# Autodesk Inventor assembly: wheel assembly
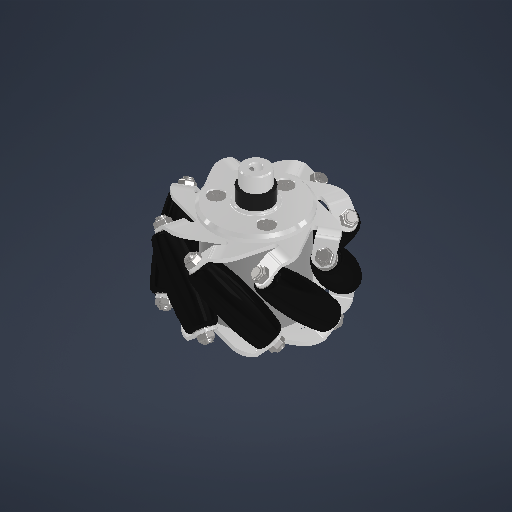
[picture p0: Inventor's stored thumbnail of the model, 512x512]
Saved by Autodesk Inventor 2025 (Build 290162000, 162)
## iProperties
Created: 2023-06-24
Part Number: wheel assembly
Document SubType Name: Assembly
Designer: khrip
Mass: 249.664 g
Surface Area: 386.365 cm^2
Volume: 54.6179 cm^3
Density: 4.5711 g/cm^3
Author: khrip
## Documents named in this file (9)
- H:\Botik\Chassis\UnsprungUnits\Wheels\wheel assembly.iam
- H:\Botik\Chassis\UnsprungUnits\Wheels\Parts\wheelHub.ipt
- H:\Botik\Chassis\UnsprungUnits\Wheels\wheelAss\Mecanum_Wheel_60mm_Right_ASM_AP214.iam
- H:\Botik\Chassis\UnsprungUnits\Wheels\Parts\washer.ipt
- C:\Users\khrip\Documents\Inventor\Content Center Files\R2025\ru-RU\GOST 17475-80 (2)\Винт 2.M4-6gx40 ГОСТ 17475-80.ipt
- C:\Users\khrip\Documents\Inventor\Content Center Files\R2025\ru-RU\GOST 17475-80 (2)\Винт 2.M3-6gx40 ГОСТ 17475-80.ipt
- C:\Users\khrip\Documents\Inventor\Content Center Files\R2025\ru-RU\GOST 11371-78  A\Шайба 3 ГОСТ 11371-78.ipt
- C:\Users\khrip\Documents\Inventor\Content Center Files\R2025\ru-RU\DIN 985\DIN 985 - M3.ipt
- H:\Botik\Chassis\UnsprungUnits\Wheels\Parts\fittingRingInstalled.ipt
## Components (14 placed, 8 different names)
1. wheelHub:1 — Совмещение:1, Совмещение:2, Совмещение:3, Совмещение:8, Совмещение:9, Совмещение:10, Совмещение:24, Совмещение:25
2. Mecanum_Wheel_60mm_Right_ASM_AP214:2 [sub-assembly] — Совмещение:1, Совмещение:2, Совмещение:3, Совмещение:4, Совмещение:5, Совмещение:6, Совмещение:12, Совмещение:14, Совмещение:16
3. washer:1 — Совмещение:4, Совмещение:5, Совмещение:6, Совмещение:7
4. Винт 2 ГОСТ 17475-80 M4 x 40:1 — Совмещение:7
5. Винт 2 ГОСТ 17475-80 M3 x 40:1 — Совмещение:8, Совмещение:13, Совмещение:19
6. Винт 2 ГОСТ 17475-80 M3 x 40:2 — Совмещение:9, Совмещение:11, Совмещение:21
7. Винт 2 ГОСТ 17475-80 M3 x 40:3 — Совмещение:10, Совмещение:15, Совмещение:17
8. Шайба  ГОСТ 11371-78 3,2:1 — Совмещение:11, Совмещение:12, Совмещение:22
9. Шайба  ГОСТ 11371-78 3,2:2 — Совмещение:13, Совмещение:14, Совмещение:20
10. Шайба  ГОСТ 11371-78 3,2:3 — Совмещение:15, Совмещение:16, Совмещение:18
11. DIN 985 - заменено на DIN EN ISO 10511 M3:1 — Совмещение:17, Совмещение:18
12. DIN 985 - заменено на DIN EN ISO 10511 M3:2 — Совмещение:19, Совмещение:20
13. DIN 985 - заменено на DIN EN ISO 10511 M3:3 — Совмещение:21, Совмещение:22
14. fittingRingInstalled:1 — Совмещение:24, Совмещение:25
## Relationships (24: Mate 24)
- Совмещение:1 [Mate]: wheelHub:1 ↔ Mecanum_Wheel_60mm_Right_ASM_AP214:2
- Совмещение:2 [Mate]: wheelHub:1 ↔ Mecanum_Wheel_60mm_Right_ASM_AP214:2
- Совмещение:3 [Mate]: wheelHub:1 ↔ Mecanum_Wheel_60mm_Right_ASM_AP214:2
- Совмещение:4 [Mate]: Mecanum_Wheel_60mm_Right_ASM_AP214:2 ↔ washer:1
- Совмещение:5 [Mate]: Mecanum_Wheel_60mm_Right_ASM_AP214:2 ↔ washer:1
- Совмещение:6 [Mate]: Mecanum_Wheel_60mm_Right_ASM_AP214:2 ↔ washer:1
- Совмещение:7 [Mate]: washer:1 ↔ Винт 2 ГОСТ 17475-80 M4 x 40:1
- Совмещение:8 [Mate]: wheelHub:1 ↔ Винт 2 ГОСТ 17475-80 M3 x 40:1
- Совмещение:9 [Mate]: wheelHub:1 ↔ Винт 2 ГОСТ 17475-80 M3 x 40:2
- Совмещение:10 [Mate]: wheelHub:1 ↔ Винт 2 ГОСТ 17475-80 M3 x 40:3
- Совмещение:11 [Mate]: Винт 2 ГОСТ 17475-80 M3 x 40:2 ↔ Шайба  ГОСТ 11371-78 3,2:1
- Совмещение:12 [Mate]: Mecanum_Wheel_60mm_Right_ASM_AP214:2 ↔ Шайба  ГОСТ 11371-78 3,2:1
- Совмещение:13 [Mate]: Винт 2 ГОСТ 17475-80 M3 x 40:1 ↔ Шайба  ГОСТ 11371-78 3,2:2
- Совмещение:14 [Mate]: Mecanum_Wheel_60mm_Right_ASM_AP214:2 ↔ Шайба  ГОСТ 11371-78 3,2:2
- Совмещение:15 [Mate]: Винт 2 ГОСТ 17475-80 M3 x 40:3 ↔ Шайба  ГОСТ 11371-78 3,2:3
- Совмещение:16 [Mate]: Mecanum_Wheel_60mm_Right_ASM_AP214:2 ↔ Шайба  ГОСТ 11371-78 3,2:3
- Совмещение:17 [Mate]: Винт 2 ГОСТ 17475-80 M3 x 40:3 ↔ DIN 985 - заменено на DIN EN ISO 10511 M3:1
- Совмещение:18 [Mate]: Шайба  ГОСТ 11371-78 3,2:3 ↔ DIN 985 - заменено на DIN EN ISO 10511 M3:1
- Совмещение:19 [Mate]: Винт 2 ГОСТ 17475-80 M3 x 40:1 ↔ DIN 985 - заменено на DIN EN ISO 10511 M3:2
- Совмещение:20 [Mate]: Шайба  ГОСТ 11371-78 3,2:2 ↔ DIN 985 - заменено на DIN EN ISO 10511 M3:2
- Совмещение:21 [Mate]: Винт 2 ГОСТ 17475-80 M3 x 40:2 ↔ DIN 985 - заменено на DIN EN ISO 10511 M3:3
- Совмещение:22 [Mate]: Шайба  ГОСТ 11371-78 3,2:1 ↔ DIN 985 - заменено на DIN EN ISO 10511 M3:3
- Совмещение:24 [Mate]: wheelHub:1 ↔ fittingRingInstalled:1
- Совмещение:25 [Mate]: wheelHub:1 ↔ fittingRingInstalled:1
